# Autodesk Inventor assembly: HPC
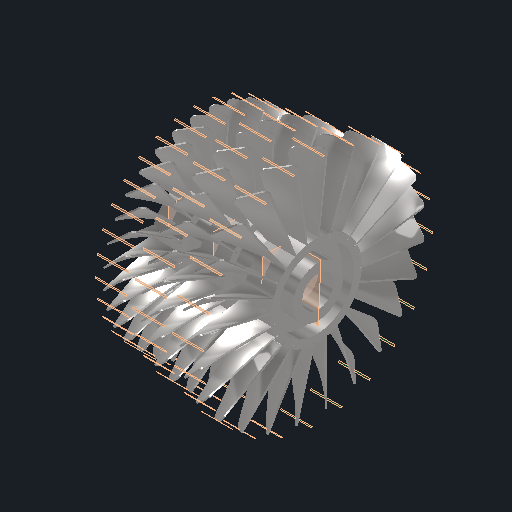
[picture p0: Inventor's stored thumbnail of the model, 512x512]
Saved by Autodesk Inventor 2026.2 (Build 302298010, 298A)
## iProperties
Created: 2026-04-26
Part Number: HPC
Document SubType Name: Assembly
Designer: Yan
Author: Yan
## Documents named in this file (6)
- C:\Users\Yan\Desktop\Turbina\HPC.iam
- C:\Users\Yan\Desktop\Turbina\Spaziamento1-2ipt.ipt
- C:\Users\Yan\Desktop\Turbina\Spaziamento2-3ipt.ipt
- C:\Users\Yan\Desktop\Turbina\Stadio1.iam
- C:\Users\Yan\Desktop\Turbina\Stadio2.iam
- C:\Users\Yan\Desktop\Turbina\Stadio3.iam
## Components (5 placed, 5 different names)
1. Spaziamento1-2ipt:1 — Mate:1, Mate:2, Mate:3
2. Spaziamento2-3ipt:1 — Mate:5, Mate:6, Mate:7
3. Stadio1:1 [sub-assembly] — Mate:1, Mate:2, Mate:4
4. Stadio2:1 [sub-assembly] — Mate:3, Mate:4, Mate:5, Mate:6, Mate:8
5. Stadio3:1 [sub-assembly] — Mate:7, Mate:8
## Relationships (8: Mate 8)
- Mate:1: Spaziamento1-2ipt:1 ↔ Stadio1:1
- Mate:2: Spaziamento1-2ipt:1 ↔ Stadio1:1
- Mate:3: Spaziamento1-2ipt:1 ↔ Stadio2:1
- Mate:4: Stadio1:1 ↔ Stadio2:1
- Mate:5: Spaziamento2-3ipt:1 ↔ Stadio2:1
- Mate:6: Spaziamento2-3ipt:1 ↔ Stadio2:1
- Mate:7: Spaziamento2-3ipt:1 ↔ Stadio3:1
- Mate:8: Stadio2:1 ↔ Stadio3:1
